# Autodesk Inventor assembly: gun 3
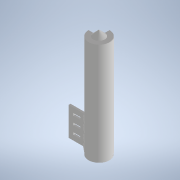
[picture p0: Inventor's stored thumbnail of the model, 180x180]
Saved by Autodesk Inventor 2020.1 (Build 241239000, 239)
## iProperties
Created: 2022-04-02
Part Number: gun 3
Document SubType Name: Assembly
Designer: User
Author: User
## Documents named in this file (8)
- D:\GitHub\TANK\3D-turret\gun 3.iam
- D:\GitHub\TANK\3D-turret\trunk.ipt
- D:\GitHub\TANK\3D-turret\barrel_holder.ipt
- D:\GitHub\TANK\3D-turret\ось пушки 3.ipt
- D:\GitHub\TANK\3D-turret\подшипник.ipt
- D:\GitHub\TANK\3D-turret\кожух пушки.ipt
- D:\GitHub\TANK\3D-turret\крышка кожуха пушки.ipt
- D:\GitHub\TANK\3D-turret\крышка кожуха пушки_ЗЕРКАЛО.ipt
## Components (14 placed, 7 different names)
1. barrel_holder:1 — Жесткий:1, Жесткий:3
2. barrel_holder:2 — Жесткий:2
3. ось пушки 3:1 — Жесткий:3, Жесткий:4, Жесткий:5
4. подшипник:1 — Жесткий:4
5. подшипник:2 — Жесткий:5, Совмещение:1
6. кожух пушки:1 — Жесткий:6, Жесткий:7
7. крышка кожуха пушки:1 — Жесткий:6
8. крышка кожуха пушки_ЗЕРКАЛО:1 — Жесткий:7, Совмещение:1
9. trunk:1 — Жесткий:1
10. trunk:2
11. trunk:3 — Жесткий:2
12. trunk:4
13. trunk:5
14. trunk:6
## Component patterns: (6 elements, first: trunk:1)
## Relationships (8: WeldJoint 7, Mate 1)
- Жесткий:1 [WeldJoint]: barrel_holder:1 ↔ trunk:1
- Жесткий:2 [WeldJoint]: barrel_holder:2 ↔ trunk:3
- Жесткий:3 [WeldJoint]: barrel_holder:1 ↔ ось пушки 3:1
- Жесткий:4 [WeldJoint]: ось пушки 3:1 ↔ подшипник:1
- Жесткий:5 [WeldJoint]: ось пушки 3:1 ↔ подшипник:2
- Жесткий:6 [WeldJoint]: кожух пушки:1 ↔ крышка кожуха пушки:1
- Жесткий:7 [WeldJoint]: кожух пушки:1 ↔ крышка кожуха пушки_ЗЕРКАЛО:1
- Совмещение:1 [Mate]: подшипник:2 ↔ крышка кожуха пушки_ЗЕРКАЛО:1
